# Autodesk Inventor assembly: 200-ROCKER-BOGIE-ASM-02
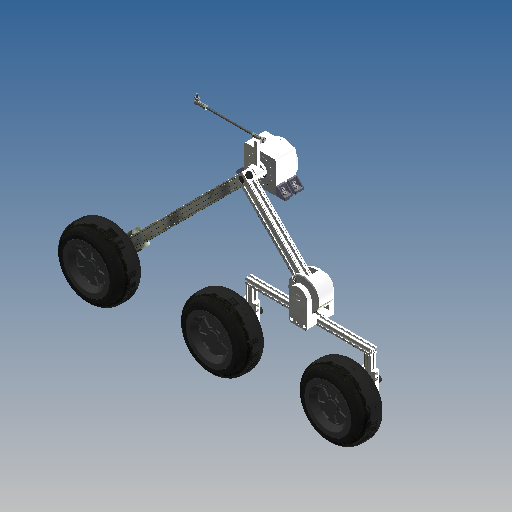
[picture p0: Inventor's stored thumbnail of the model, 512x512]
Saved by Autodesk Inventor 2018.2 (Build 222227000, 227)
## iProperties
Manager: feesmrt
Company: FRANC0R
Created: 2017-12-10
Part Number: 200-ROCKER-BOGIE-ASM-02
Material: Generisch
Document SubType Name: Assembly
Designer: feesmrt
Project: Rescue Robot
Description: Rocker Bogie Suspension
Engineer: feesmrt
Authority: feesmrt
Stock Number: 200-ROCKER-BOGIE-ASM
Author: feesmrt
Title: Rocker Bogie Suspension
Subject: Rescue Robot
Revision Number: 1
## Documents named in this file (5)
- D:\Programmierung\FRANC0R\CAD\02-Rocker-Bogie-Robot\200-ROCKER-BOGIE\200-ROCKER-BOGIE-ASM-02.iam
- D:\Programmierung\FRANC0R\CAD\02-Rocker-Bogie-Robot\200-ROCKER-BOGIE\200-50-WHEEL-CONNECTOR\200-50-WHEEL-CONNECTOR-20MM-ASM-01.iam
- D:\Programmierung\FRANC0R\CAD\02-Rocker-Bogie-Robot\200-ROCKER-BOGIE\200-50-WHEEL-CONNECTOR\200-50-WHEEL-CONNECTOR-30MM-ASM-01.iam
- D:\Programmierung\FRANC0R\CAD\02-Rocker-Bogie-Robot\200-ROCKER-BOGIE\200-ROCKER-ASM-02.iam
- D:\Programmierung\FRANC0R\CAD\02-Rocker-Bogie-Robot\200-ROCKER-BOGIE\200-BOGIE-ASM-02.iam
## Components (5 placed, 4 different names)
1. 200-ROCKER-ASM-02:1 [sub-assembly] — Passend:1, Passend:2, Passend:3, Passend:4, Fluchtend:1, Passend:5
2. 200-BOGIE-ASM-02:1 [sub-assembly] — Passend:1, Passend:2, Passend:3, Passend:6, Fluchtend:2, Passend:7, Passend:8, Passend:9, Fluchtend:3
3. 200-50-WHEEL-CONNECTOR-20MM-ASM-01:1 [sub-assembly] — Passend:6, Fluchtend:2, Passend:7
4. 200-50-WHEEL-CONNECTOR-20MM-ASM-01:2 [sub-assembly] — Passend:8, Passend:9, Fluchtend:3
5. 200-50-WHEEL-CONNECTOR-30MM-ASM-01:1 [sub-assembly] — Passend:4, Fluchtend:1, Passend:5
## Relationships (12: Mate 9, Flush 3)
- Passend:1 [Mate]: 200-ROCKER-ASM-02:1 ↔ 200-BOGIE-ASM-02:1
- Passend:2 [Mate]: 200-ROCKER-ASM-02:1 ↔ 200-BOGIE-ASM-02:1
- Passend:3 [Mate]: 200-ROCKER-ASM-02:1 ↔ 200-BOGIE-ASM-02:1
- Passend:4 [Mate]: 200-ROCKER-ASM-02:1 ↔ 200-50-WHEEL-CONNECTOR-30MM-ASM-01:1
- Fluchtend:1 [Flush]: 200-ROCKER-ASM-02:1 ↔ 200-50-WHEEL-CONNECTOR-30MM-ASM-01:1
- Passend:5 [Mate]: 200-ROCKER-ASM-02:1 ↔ 200-50-WHEEL-CONNECTOR-30MM-ASM-01:1
- Passend:6 [Mate]: 200-BOGIE-ASM-02:1 ↔ 200-50-WHEEL-CONNECTOR-20MM-ASM-01:1
- Fluchtend:2 [Flush]: 200-BOGIE-ASM-02:1 ↔ 200-50-WHEEL-CONNECTOR-20MM-ASM-01:1
- Passend:7 [Mate]: 200-BOGIE-ASM-02:1 ↔ 200-50-WHEEL-CONNECTOR-20MM-ASM-01:1
- Passend:8 [Mate]: 200-BOGIE-ASM-02:1 ↔ 200-50-WHEEL-CONNECTOR-20MM-ASM-01:2
- Passend:9 [Mate]: 200-BOGIE-ASM-02:1 ↔ 200-50-WHEEL-CONNECTOR-20MM-ASM-01:2
- Fluchtend:3 [Flush]: 200-BOGIE-ASM-02:1 ↔ 200-50-WHEEL-CONNECTOR-20MM-ASM-01:2
